# Autodesk Inventor assembly: LoadCellSupport
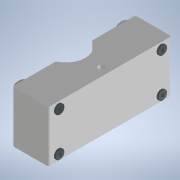
[picture p0: Inventor's stored thumbnail of the model, 180x180]
Saved by Autodesk Inventor 2022 (Build 260153000, 153)
## iProperties
Created: 2021-11-09
Part Number: LoadCellSupport
Document SubType Name: Assembly
Designer: JK
Author: JK
## Documents named in this file (4)
- C:\Users\JK\Documents\Inventor\UTM\LoadCellSupport.iam
- C:\Users\JK\Documents\Inventor\UTM\LowerSupport.ipt
- C:\Users\JK\Documents\Inventor\UTM\PernoM5x40Plano.ipt
- C:\Users\JK\Documents\Inventor\UTM\TuercaTM5Perfil2020.ipt
## Components (9 placed, 3 different names)
1. LowerSupport:1 — Coincidencia:2, Ángulo:1, Coincidencia:4
2. PernoM5x40Plano:1 — Coincidencia:2, Coincidencia:3
3. TuercaTM5Perfil2020:1 — Coincidencia:3, Ángulo:1, Coincidencia:4
4. PernoM5x40Plano:2
5. TuercaTM5Perfil2020:2
6. PernoM5x40Plano:3
7. TuercaTM5Perfil2020:3
8. PernoM5x40Plano:4
9. TuercaTM5Perfil2020:4
## Component patterns: (4 elements, first: PernoM5x40Plano:1 + TuercaTM5Perfil2020:1)
## Relationships (5: Mate 4, Angle 1)
- [Mate]: LowerSupport:1 ↔ PernoM5x40Plano:1
- Coincidencia:2 [Mate]: LowerSupport:1 ↔ PernoM5x40Plano:1
- Coincidencia:3 [Mate]: PernoM5x40Plano:1 ↔ TuercaTM5Perfil2020:1
- Ángulo:1 [Angle] (0 deg): LowerSupport:1 ↔ TuercaTM5Perfil2020:1
- Coincidencia:4 [Mate] (0.7 mm): LowerSupport:1 ↔ TuercaTM5Perfil2020:1
